# Autodesk Inventor assembly: arm of robot
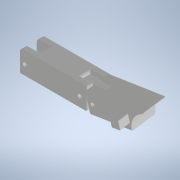
[picture p0: Inventor's stored thumbnail of the model, 180x180]
Saved by Autodesk Inventor 2022 (Build 260153000, 153)
## iProperties
Created: 2021-07-21
Part Number: arm of robot
Document SubType Name: Assembly
Designer: fanam
Author: fanam
## Documents named in this file (4)
- C:\Users\fanam\OneDrive\سطح المكتب\arm of robot.iam
- C:\Users\fanam\OneDrive\سطح المكتب\engin part1.ipt
- C:\Users\fanam\OneDrive\سطح المكتب\the arm part 1.ipt
- C:\Users\fanam\OneDrive\سطح المكتب\the arm part 2.ipt
## Components (3 placed, 3 different names)
1. engin part1:1 — Mate:1, Mate:2
2. the arm part 1:1 — Mate:1
3. the arm part 2:1 — Mate:2
## Relationships (2: Mate 2)
- Mate:1: engin part1:1 ↔ the arm part 1:1
- Mate:2: engin part1:1 ↔ the arm part 2:1
